# Autodesk Inventor assembly: Gesamtansicht
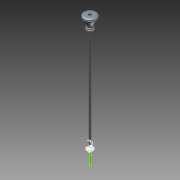
[picture p0: Inventor's stored thumbnail of the model, 180x180]
Saved by Autodesk Inventor 2012 (Build 160160000, 160)
## iProperties
Created: 2014-06-24
Part Number: Gesamtansicht
Document SubType Name: Assembly
Designer: kathrin.ganzhorn
Author: kathrin.ganzhorn
## Documents named in this file (14)
- \\wmi\user\groups\Magnetiker\Maier-Flaig\2014-09 Flexline-Probenstab\1-autodesk project\assembly.iam
- \\wmi\user\groups\Magnetiker\Maier-Flaig\2014-09 Flexline-Probenstab\1-autodesk project\v2a-tube.ipt
- \\wmi\user\groups\Magnetiker\Maier-Flaig\2014-09 Flexline-Probenstab\1-autodesk project\Importierte Komponenten\110FBL016\110FBL016.ipt
- \\wmi\user\groups\Magnetiker\Maier-Flaig\2014-09 Flexline-Probenstab\1-autodesk project\Importierte Komponenten\116ZRG016\116ZRG016.ipt
- \\wmi\user\groups\Magnetiker\Maier-Flaig\2014-09 Flexline-Probenstab\1-autodesk project\PEEK-extension.ipt
- PEEK-extension.ipt
- \\wmi\user\groups\Magnetiker\Maier-Flaig\2014-09 Flexline-Probenstab\1-autodesk project\PEEK-PCB-holder.ipt
- \\wmi\user\groups\Magnetiker\Maier-Flaig\2014-09 Flexline-Probenstab\1-autodesk project\PCB.ipt
- \\wmi\user\groups\Magnetiker\Maier-Flaig\2014-09 Flexline-Probenstab\1-autodesk project\pin_socket.ipt
- \\wmi\user\groups\Magnetiker\Maier-Flaig\2014-09 Flexline-Probenstab\1-autodesk project\resonator.ipt
- \\wmi\user\groups\Magnetiker\Maier-Flaig\2014-09 Flexline-Probenstab\1-autodesk project\pin_header.ipt
- \\wmi\user\groups\Magnetiker\Maier-Flaig\2014-09 Flexline-Probenstab\1-autodesk project\Importierte Komponenten\116ZRG040\116ZRG040.ipt
- \\wmi\user\groups\Magnetiker\Maier-Flaig\2014-09 Flexline-Probenstab\1-autodesk project\Importierte Komponenten\120RRK040-016-40\120RRK040-016-40.ipt
- \\wmi\user\groups\Magnetiker\Maier-Flaig\2014-09 Flexline-Probenstab\1-autodesk project\Importierte Komponenten\110FBL040\110FBL040.ipt
## Components (12 placed, 12 different names)
1. v2a-tube:1 — Einfügen:2, Einfügen:11, Einfügen:14
2. Pfeiffer-KF16-Blindflansch — Einfügen:2, Einfügen:3
3. Pfeiffer-KF16-Zentrierring — Einfügen:3, Einfügen:16
4. PEEK-extension:1 — Einfügen:11
5. PCB:1 — Einfügen:13, Passend:1, Passend:4, Passend:5, Passend:6, Passend:7, Passend:8
6. PEEK-PCB-holder:2 — Einfügen:13, Einfügen:14, Passend:1, Einfügen:15
7. pin_socket:1 — Passend:6, Passend:7, Passend:8
8. resonator:1 — Einfügen:15
9. pin_header:1 — Passend:4, Passend:5
10. 120RRK040-016-40:1 — Einfügen:16, Einfügen:17
11. 116ZRG040:1 — Einfügen:17, Einfügen:18
12. 110FBL040:1 — Einfügen:18
## Relationships (15: Insert 9, Mate 6)
- Einfügen:2 [Insert]: v2a-tube:1 ↔ Pfeiffer-KF16-Blindflansch
- Einfügen:3 [Insert]: Pfeiffer-KF16-Blindflansch ↔ Pfeiffer-KF16-Zentrierring
- Einfügen:11 [Insert]: v2a-tube:1 ↔ PEEK-extension:1
- Einfügen:13 [Insert]: PCB:1 ↔ PEEK-PCB-holder:2
- Einfügen:14 [Insert]: v2a-tube:1 ↔ PEEK-PCB-holder:2
- Passend:1 [Mate]: PCB:1 ↔ PEEK-PCB-holder:2
- Einfügen:15 [Insert]: PEEK-PCB-holder:2 ↔ resonator:1
- Passend:4 [Mate]: PCB:1 ↔ pin_header:1
- Passend:5 [Mate] (-5 mm): PCB:1 ↔ pin_header:1
- Passend:6 [Mate]: PCB:1 ↔ pin_socket:1
- Passend:7 [Mate]: PCB:1 ↔ pin_socket:1
- Passend:8 [Mate]: PCB:1 ↔ pin_socket:1
- Einfügen:16 [Insert]: Pfeiffer-KF16-Zentrierring ↔ 120RRK040-016-40:1
- Einfügen:17 [Insert]: 120RRK040-016-40:1 ↔ 116ZRG040:1
- Einfügen:18 [Insert]: 116ZRG040:1 ↔ 110FBL040:1
